# Autodesk Inventor assembly: Chessboard Design
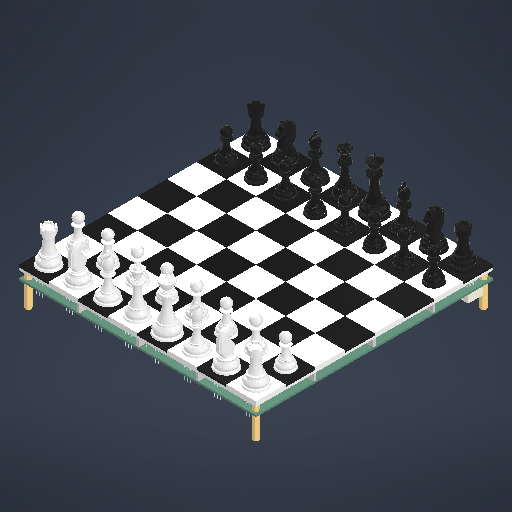
[picture p0: Inventor's stored thumbnail of the model, 512x512]
Saved by Autodesk Inventor 2026 (Build 300175000, 175)
## iProperties
Created: 2025-04-19
Part Number: Chessboard Design
Document SubType Name: Assembly
Designer: ckyiu
Author: ckyiu
## Documents named in this file (16)
- C:\Users\ckyiu\Documents\Projects\Chessboard-Design\Chessboard Design.iam
- C:\Users\ckyiu\Documents\Projects\Chessboard-Design\Assemblies\Chessboard Bottom.iam
- C:\Users\ckyiu\Documents\Projects\Chessboard-Design\Parts\Square Holder Support.ipt
- C:\Users\ckyiu\Documents\Projects\Chessboard-Design\Assemblies\Chessboard Top.iam
- C:\Users\ckyiu\Documents\Projects\Chessboard-Design\Assemblies\Chess Pieces\White Pawn.iam
- C:\Users\ckyiu\Documents\Projects\Chessboard-Design\Assemblies\Chess Pieces\White Rook.iam
- C:\Users\ckyiu\Documents\Projects\Chessboard-Design\Assemblies\Chess Pieces\White Knight.iam
- C:\Users\ckyiu\Documents\Projects\Chessboard-Design\Assemblies\Chess Pieces\White Bishop.iam
- C:\Users\ckyiu\Documents\Projects\Chessboard-Design\Assemblies\Chess Pieces\White Queen.iam
- C:\Users\ckyiu\Documents\Projects\Chessboard-Design\Assemblies\Chess Pieces\White King.iam
- C:\Users\ckyiu\Documents\Projects\Chessboard-Design\Assemblies\Chess Pieces\Black Pawn.iam
- C:\Users\ckyiu\Documents\Projects\Chessboard-Design\Assemblies\Chess Pieces\Black Rook.iam
- C:\Users\ckyiu\Documents\Projects\Chessboard-Design\Assemblies\Chess Pieces\Black Knight.iam
- C:\Users\ckyiu\Documents\Projects\Chessboard-Design\Assemblies\Chess Pieces\Black Bishop.iam
- C:\Users\ckyiu\Documents\Projects\Chessboard-Design\Assemblies\Chess Pieces\Black Queen.iam
- C:\Users\ckyiu\Documents\Projects\Chessboard-Design\Assemblies\Chess Pieces\Black King.iam
## Components (35 placed, 15 different names)
1. Chessboard Bottom:1 [sub-assembly] — Mate:1, Flush:1, Flush:2, Flush:3, Flush:4
2. Square Holder Support:1 — Mate:1, Flush:1, Flush:2, Mate:2
3. Chessboard Top:1 [sub-assembly] — Mate:2, Flush:3, Flush:4, Rigid:1, Rigid:2, Rigid:3, Rigid:4, Rigid:5, Rigid:6, Rigid:7, Rigid:8, Rigid:9, Rigid:10, Rigid:11, Rigid:12, Rigid:13, Rigid:14, Rigid:15, Rigid:16, Rigid:17, Rigid:18
4. White Rook:1 [sub-assembly] — Rigid:2
5. White Rook:2 [sub-assembly] — Rigid:3
6. White Knight:1 [sub-assembly] — Rigid:4
7. White Knight:2 [sub-assembly] — Rigid:5
8. White Bishop:1 [sub-assembly] — Rigid:6
9. White Bishop:2 [sub-assembly] — Rigid:7
10. White Queen:1 [sub-assembly] — Rigid:8
11. White King:1 [sub-assembly] — Rigid:9
12. Black Rook:1 [sub-assembly] — Rigid:11
13. Black Rook:2 [sub-assembly] — Rigid:12
14. Black Knight:1 [sub-assembly] — Rigid:14
15. Black Knight:2 [sub-assembly] — Rigid:13
16. Black Bishop:1 [sub-assembly] — Rigid:15
17. Black Bishop:2 [sub-assembly] — Rigid:16
18. Black Queen:1 [sub-assembly] — Rigid:17
19. Black King:1 [sub-assembly] — Rigid:18
20. White Pawn:1 [sub-assembly] — Rigid:1
21. White Pawn:2 [sub-assembly]
22. White Pawn:3 [sub-assembly]
23. White Pawn:4 [sub-assembly]
24. White Pawn:5 [sub-assembly]
25. White Pawn:6 [sub-assembly]
26. White Pawn:7 [sub-assembly]
27. White Pawn:8 [sub-assembly]
28. Black Pawn:1 [sub-assembly] — Rigid:10
29. Black Pawn:2 [sub-assembly]
30. Black Pawn:3 [sub-assembly]
31. Black Pawn:4 [sub-assembly]
32. Black Pawn:5 [sub-assembly]
33. Black Pawn:6 [sub-assembly]
34. Black Pawn:7 [sub-assembly]
35. Black Pawn:8 [sub-assembly]
## Component patterns: (8 elements, first: White Pawn:1), (8 elements, first: Black Pawn:1)
## Relationships (24: WeldJoint 18, Flush 4, Mate 2)
- Mate:1: Chessboard Bottom:1 ↔ Square Holder Support:1
- Flush:1: Chessboard Bottom:1 ↔ Square Holder Support:1
- Flush:2: Chessboard Bottom:1 ↔ Square Holder Support:1
- Mate:2: Square Holder Support:1 ↔ Chessboard Top:1
- Flush:3: Chessboard Bottom:1 ↔ Chessboard Top:1
- Flush:4: Chessboard Bottom:1 ↔ Chessboard Top:1
- Rigid:1 [WeldJoint]: Chessboard Top:1 ↔ White Pawn:1
- Rigid:2 [WeldJoint]: Chessboard Top:1 ↔ White Rook:1
- Rigid:3 [WeldJoint]: Chessboard Top:1 ↔ White Rook:2
- Rigid:4 [WeldJoint]: Chessboard Top:1 ↔ White Knight:1
- Rigid:5 [WeldJoint]: Chessboard Top:1 ↔ White Knight:2
- Rigid:6 [WeldJoint]: Chessboard Top:1 ↔ White Bishop:1
- Rigid:7 [WeldJoint]: Chessboard Top:1 ↔ White Bishop:2
- Rigid:8 [WeldJoint]: Chessboard Top:1 ↔ White Queen:1
- Rigid:9 [WeldJoint]: Chessboard Top:1 ↔ White King:1
- Rigid:10 [WeldJoint]: Chessboard Top:1 ↔ Black Pawn:1
- Rigid:11 [WeldJoint]: Chessboard Top:1 ↔ Black Rook:1
- Rigid:12 [WeldJoint]: Chessboard Top:1 ↔ Black Rook:2
- Rigid:13 [WeldJoint]: Chessboard Top:1 ↔ Black Knight:2
- Rigid:14 [WeldJoint]: Chessboard Top:1 ↔ Black Knight:1
- Rigid:15 [WeldJoint]: Chessboard Top:1 ↔ Black Bishop:1
- Rigid:16 [WeldJoint]: Chessboard Top:1 ↔ Black Bishop:2
- Rigid:17 [WeldJoint]: Chessboard Top:1 ↔ Black Queen:1
- Rigid:18 [WeldJoint]: Chessboard Top:1 ↔ Black King:1
